# Autodesk Inventor assembly: 조립품1
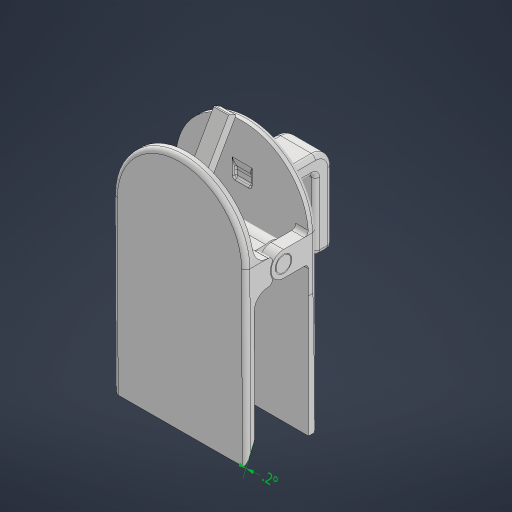
[picture p0: Inventor's stored thumbnail of the model, 512x512]
Saved by Autodesk Inventor 2024 (Build 280153000, 153)
## iProperties
Created: 2024-01-27
Part Number: 조립품1
Document SubType Name: Assembly
Designer: likek
Author: likek
## Documents named in this file (4)
- D:\github\Modeling\IKEA 페그보드 시제품\조립품1.iam
- D:\github\Modeling\IKEA 페그보드 시제품\집게 베이스.ipt
- D:\github\Modeling\IKEA 페그보드 시제품\집게 이동.ipt
- D:\github\Modeling\IKEA 페그보드 시제품\집게 고정.ipt
## Components (3 placed, 3 different names)
1. 집게 베이스:1 — 삽입:1, 각도:2
2. 집게 이동:1 — 삽입:1, 삽입:2, 각도:1, 각도:2
3. 집게 고정:1 — 삽입:2, 각도:1
## Relationships (4: Insert 2, Angle 2)
- 삽입:1 [Insert]: 집게 베이스:1 ↔ 집게 이동:1
- 삽입:2 [Insert]: 집게 이동:1 ↔ 집게 고정:1
- 각도:1 [Angle] (150 deg): 집게 이동:1 ↔ 집게 고정:1
- 각도:2 [Angle] (180 deg): 집게 베이스:1 ↔ 집게 이동:1
